# Autodesk Inventor assembly: Assembly_Cube_Kinematic_Mirrormount_Thorlabs_90_PRO_v3
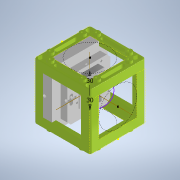
[picture p0: Inventor's stored thumbnail of the model, 180x180]
Saved by Autodesk Inventor 2022.3 (Build 263350000, 350)
## iProperties
Created: 2021-11-15
Part Number: Assembly_Cube_Kinematic_Mirrormount_Thorlabs_90_PRO_v3
Document SubType Name: Assembly
Designer: diederichbenedict
Author: diederichbenedict
## Documents named in this file (5)
- C:\Users\bingoeleda\Desktop\Modules\!! 12.Reference_Mirror_with_VCA_Module (Mirror_Kinematic_PRO_90_Module)\Assembly_Cube_Kinematic_Mirrormount_Thorlabs_90_PRO_VCA_v3.iam
- G:\My Drive\ASP - M.Sc. Photonics\Practical Modules\MODULE 4 - Master Thesis\3.Experiments\2.Michelson and OCT with UC2 system\Modules\2.Base_Cube\Base_Cube_IM\Assembly_Cube_empty_IM_v3.iam
- C:\Users\bingoeleda\Desktop\Modules\!! 12.Reference_Mirror_with_VCA_Module (Mirror_Kinematic_PRO_90_Module)\20_Cube_Insert_Kinematic_Mirror_90_pro_v3.ipt
- G:\My Drive\ASP - M.Sc. Photonics\Practical Modules\MODULE 4 - Master Thesis\3.Experiments\2.Michelson and OCT with UC2 system\Modules\!! 12.Reference_Mirror_with_VCA_Module (Mirror_Kinematic_PRO_90_Module)\20_Cube_Insert_Kinematic_Mirrormount_90_pro_v3.ipt
- C:\Users\bingoeleda\Desktop\Modules\!! 12.Reference_Mirror_with_VCA_Module (Mirror_Kinematic_PRO_90_Module)\00_KES400.iam
## Components (4 placed, 4 different names)
1. Assembly_Cube_empty_IM_v3:1 [sub-assembly] — Mate:2, Mate:3, Mate:4, Angle:1, Angle:2, Mate:5
2. 20_Cube_Insert_Kinematic_Mirror_90_pro_v3:1 — Mate:2, Mate:3, Mate:4, Angle:1, Angle:2, Mate:5, Rotational:1
3. 20_Cube_Insert_Kinematic_Mirrormount_90_pro_v3:2 — Mate:6, Mate:7, Rotational:1
4. 00_KES400:1 [sub-assembly] — Mate:6, Mate:7
## Relationships (9: Mate 6, Angle 2, RevoluteJoint 1)
- Mate:2: Assembly_Cube_empty_IM_v3:1 ↔ 20_Cube_Insert_Kinematic_Mirror_90_pro_v3:1
- Mate:3: Assembly_Cube_empty_IM_v3:1 ↔ 20_Cube_Insert_Kinematic_Mirror_90_pro_v3:1
- Mate:4: Assembly_Cube_empty_IM_v3:1 ↔ 20_Cube_Insert_Kinematic_Mirror_90_pro_v3:1
- Angle:1 (0 deg): Assembly_Cube_empty_IM_v3:1 ↔ 20_Cube_Insert_Kinematic_Mirror_90_pro_v3:1
- Angle:2 (0 deg): Assembly_Cube_empty_IM_v3:1 ↔ 20_Cube_Insert_Kinematic_Mirror_90_pro_v3:1
- Mate:5: Assembly_Cube_empty_IM_v3:1 ↔ 20_Cube_Insert_Kinematic_Mirror_90_pro_v3:1
- Mate:6: 20_Cube_Insert_Kinematic_Mirrormount_90_pro_v3:2 ↔ 00_KES400:1
- Mate:7: 20_Cube_Insert_Kinematic_Mirrormount_90_pro_v3:2 ↔ 00_KES400:1
- Rotational:1 [RevoluteJoint] (-2 mm): 20_Cube_Insert_Kinematic_Mirror_90_pro_v3:1 ↔ 20_Cube_Insert_Kinematic_Mirrormount_90_pro_v3:2
